# Autodesk Inventor assembly: Final
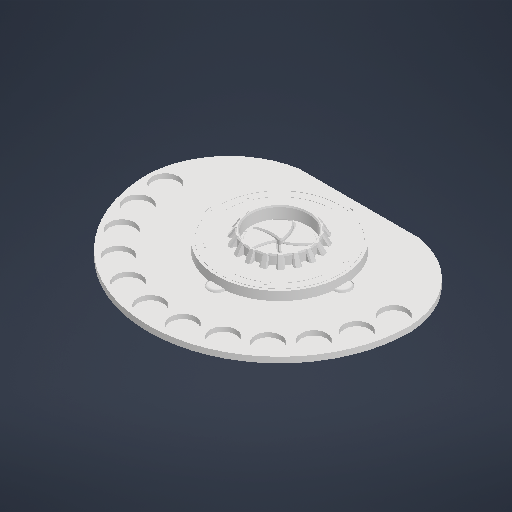
[picture p0: Inventor's stored thumbnail of the model, 512x512]
Saved by Autodesk Inventor 2026.2 (Build 302298000, 298)
## iProperties
Created: 2025-12-31
Part Number: Final
Document SubType Name: Assembly
Designer: Cobble
Author: Cobble
## Documents named in this file (3)
- D:\CAD\Final.iam
- D:\CAD\Shot FIller V2\BasePlate.ipt
- D:\CAD\Shot FIller V2\Aperatus 100mm\Aperatus.iam
## Components (2 placed, 2 different names)
1. BasePlate:1 — Insert:1, Insert:2, Insert:3
2. Aperatus:1 [sub-assembly] — Insert:1, Insert:2, Insert:3
## Relationships (3: Insert 3)
- Insert:1: BasePlate:1 ↔ Aperatus:1
- Insert:2: BasePlate:1 ↔ Aperatus:1
- Insert:3: BasePlate:1 ↔ Aperatus:1
